# Autodesk Inventor assembly: Concept 3 Assembly
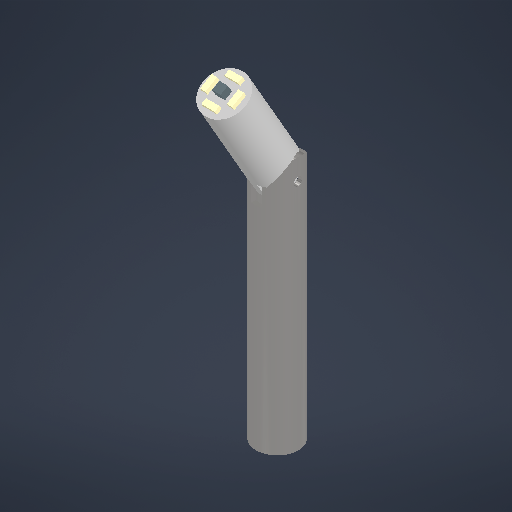
[picture p0: Inventor's stored thumbnail of the model, 512x512]
Saved by Autodesk Inventor 2026.2 (Build 302298010, 298A)
## iProperties
Created: 2026-04-02
Part Number: Concept 3 Assembly
Document SubType Name: Assembly
Designer: piete
Author: piete
## Documents named in this file (5)
- C:\Users\piete\Desktop\Skripsie\Documents\Concept Designs\Concept 3 1 Degree of Freedom\Concept 3 Assembly.iam
- C:\Users\piete\Desktop\Skripsie\Documents\Concept Designs\Concept 3 1 Degree of Freedom\Shaft.ipt
- C:\Users\piete\Desktop\Skripsie\Documents\Concept Designs\Concept 3 1 Degree of Freedom\Camera encase.ipt
- C:\Users\piete\Desktop\Skripsie\Documents\Concept Designs\Camera sensor.ipt
- C:\Users\piete\Desktop\Skripsie\Documents\Concept Designs\Large light.ipt
## Components (7 placed, 4 different names)
1. Shaft:1 — Mate:1, Flush:1, Angle:1
2. Camera encase:1 — Mate:1, Flush:1, Angle:1, Mate:2, Flush:2, Flush:3, Mate:4, Mate:5, Mate:7, Mate:8, Mate:9, Flush:4, Flush:5, Mate:10, Mate:11, Mate:12, Flush:6, Mate:13
3. Camera sensor:1 — Mate:2, Flush:2, Flush:3
4. Large light:1 — Mate:4, Mate:11, Flush:6
5. Large light:3 — Mate:8, Flush:4, Flush:5
6. Large light:4 — Mate:7, Mate:9, Mate:10
7. Large light:5 — Mate:5, Mate:12, Mate:13
## Relationships (18: Mate 11, Flush 6, Angle 1)
- Mate:1: Shaft:1 ↔ Camera encase:1
- Flush:1: Shaft:1 ↔ Camera encase:1
- Angle:1 (-30 deg): Shaft:1 ↔ Camera encase:1
- Mate:2: Camera encase:1 ↔ Camera sensor:1
- Flush:2 (-1 mm): Camera encase:1 ↔ Camera sensor:1
- Flush:3 (-1 mm): Camera encase:1 ↔ Camera sensor:1
- Mate:4: Camera encase:1 ↔ Large light:1
- Mate:5: Camera encase:1 ↔ Large light:5
- Mate:7: Camera encase:1 ↔ Large light:4
- Mate:8: Camera encase:1 ↔ Large light:3
- Mate:9 (2.5 mm): Camera encase:1 ↔ Large light:4
- Flush:4 (2.5 mm): Camera encase:1 ↔ Large light:3
- Flush:5: Camera encase:1 ↔ Large light:3
- Mate:10: Camera encase:1 ↔ Large light:4
- Mate:11: Camera encase:1 ↔ Large light:1
- Mate:12: Camera encase:1 ↔ Large light:5
- Flush:6 (2.5 mm): Camera encase:1 ↔ Large light:1
- Mate:13 (2.5 mm): Camera encase:1 ↔ Large light:5
